# Autodesk Inventor assembly: 28-35-001
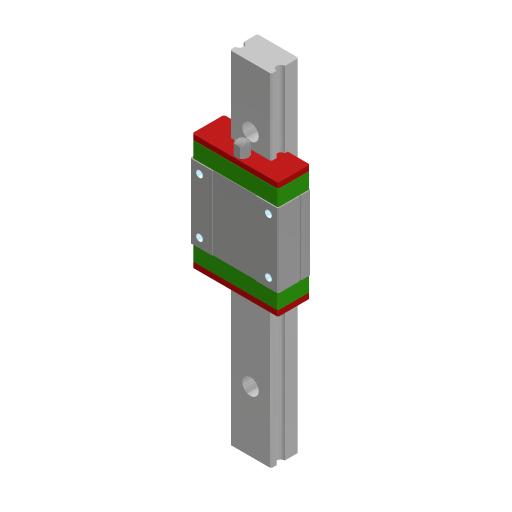
[picture p0: Inventor's stored thumbnail of the model, 512x512]
Saved by Autodesk Inventor 2023 (Build 270158000, 158)
## iProperties
Created: 2026-04-09
Part Number: 28-35-001
Document SubType Name: Assembly
Designer: ferrerx
Author: ferrerx
Revision Number: ANYUNSPECIFIED
## Documents named in this file (3)
- C:\Users\ferrerx\The Francis Crick Dropbox\MakingLab\Projects\MSTP00412 - Linear cell stretcher\28-35-001.iam
- C:\Users\ferrerx\The Francis Crick Dropbox\MakingLab\Projects\MSTP00412 - Linear cell stretcher\28-35-002.ipt
- C:\Users\ferrerx\The Francis Crick Dropbox\MakingLab\Projects\MSTP00412 - Linear cell stretcher\28-42-903.ipt
## Components (2 placed, 2 different names)
1. 28-35-002 — Mate:1, Mate:2, Flush:1
2. 28-42-903 — Mate:1, Mate:2, Flush:1
## Relationships (3: Mate 2, Flush 1)
- Mate:1: 28-35-002 ↔ 28-42-903
- Mate:2: 28-35-002 ↔ 28-42-903
- Flush:1 (27.45 mm): 28-35-002 ↔ 28-42-903
